# Autodesk Inventor assembly: złożenie
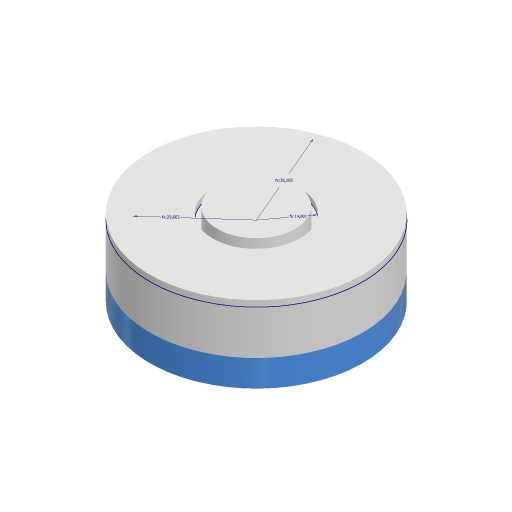
[picture p0: Inventor's stored thumbnail of the model, 512x512]
Saved by Autodesk Inventor 2024 (Build 280153000, 153)
## iProperties
Created: 2024-12-22
Part Number: złożenie
Document SubType Name: Assembly
Designer: Wicek
Author: Wicek
## Documents named in this file (8)
- I:\Dyski współdzielone\skill.ed TaskHunter\Model 3D\Przekładnia cykloidalna\złożenie.iam
- I:\Dyski współdzielone\skill.ed TaskHunter\Model 3D\Przekładnia cykloidalna\Korpus.ipt
- C:\Users\Wicek\OneDrive\Dokumenty\Inventor\Content Center Files\R2024\pl-PL\BS 290 SKF(09)\BS 290 SKF - SKF 608-2Z.ipt
- I:\Dyski współdzielone\skill.ed TaskHunter\Model 3D\Przekładnia cykloidalna\Dysk_we.ipt
- I:\Dyski współdzielone\skill.ed TaskHunter\Model 3D\Przekładnia cykloidalna\rotor.ipt
- I:\Dyski współdzielone\skill.ed TaskHunter\Model 3D\Przekładnia cykloidalna\Dysk_wy.ipt
- I:\Dyski współdzielone\skill.ed TaskHunter\Model 3D\Przekładnia cykloidalna\Korpus 2.ipt
- I:\Dyski współdzielone\skill.ed TaskHunter\Model 3D\Przekładnia cykloidalna\parametry.xlsx
## Components (7 placed, 6 different names)
1. Korpus:1 — Zestawiające:1, Zestawiające:4, Zestawiające:14
2. BS 290 SKF- osłonięte obustronnie SKF 608-2Z:1 — Zestawiające:2, Zestawiające:3, Równoległe:2, Zestawiające:4, Zestawiające:11, Zestawiające:12
3. Dysk_we:1 — Zestawiające:2, Zestawiające:1, Obrót:1, Zestawiające:6, Zestawiające:7, Zestawiające:12
4. rotor:1 — Zestawiające:3, Równoległe:2, Obrót:1, Obrót:2
5. Dysk_wy:1 — Zestawiające:8, Zestawiające:9, Zestawiające:10, Obrót:2, Zestawiające:13
6. BS 290 SKF- osłonięte obustronnie SKF 608-2Z:2 — Zestawiające:6, Zestawiające:7, Zestawiające:8, Zestawiające:9, Zestawiające:10, Zestawiające:11
7. Korpus 2:1 — Zestawiające:13, Zestawiające:14
## Relationships (16: Mate 13, RelateRotation 2, Flush 1)
- Zestawiające:1 [Mate]: Korpus:1 ↔ Dysk_we:1
- Zestawiające:2 [Mate]: BS 290 SKF- osłonięte obustronnie SKF 608-2Z:1 ↔ Dysk_we:1
- Zestawiające:3 [Mate]: BS 290 SKF- osłonięte obustronnie SKF 608-2Z:1 ↔ rotor:1
- Równoległe:2 [Flush]: BS 290 SKF- osłonięte obustronnie SKF 608-2Z:1 ↔ rotor:1
- Zestawiające:4 [Mate]: Korpus:1 ↔ BS 290 SKF- osłonięte obustronnie SKF 608-2Z:1
- Obrót:1 [RelateRotation] (0.0312 ul): Dysk_we:1 ↔ rotor:1
- Zestawiające:6 [Mate]: Dysk_we:1 ↔ BS 290 SKF- osłonięte obustronnie SKF 608-2Z:2
- Zestawiające:7 [Mate]: Dysk_we:1 ↔ BS 290 SKF- osłonięte obustronnie SKF 608-2Z:2
- Zestawiające:8 [Mate]: Dysk_wy:1 ↔ BS 290 SKF- osłonięte obustronnie SKF 608-2Z:2
- Zestawiające:9 [Mate]: Dysk_wy:1 ↔ BS 290 SKF- osłonięte obustronnie SKF 608-2Z:2
- Zestawiające:10 [Mate]: Dysk_wy:1 ↔ BS 290 SKF- osłonięte obustronnie SKF 608-2Z:2
- Zestawiające:11 [Mate]: BS 290 SKF- osłonięte obustronnie SKF 608-2Z:1 ↔ BS 290 SKF- osłonięte obustronnie SKF 608-2Z:2
- Obrót:2 [RelateRotation] (1 ul): rotor:1 ↔ Dysk_wy:1
- Zestawiające:12 [Mate]: BS 290 SKF- osłonięte obustronnie SKF 608-2Z:1 ↔ Dysk_we:1
- Zestawiające:13 [Mate]: Dysk_wy:1 ↔ Korpus 2:1
- Zestawiające:14 [Mate]: Korpus:1 ↔ Korpus 2:1
## Named parameters: Lrz = 11 mm, Lrw = 4 mm, Lh = 7 mm, N1 = 31, N2 = 6, Rr = 1.5 mm, R = 29.60282 mm, R1 = 5 mm, h1 = 2 mm, h2 = 5 mm, E1 = 0.75 mm, silnik_rw = 2.5 mm, silnik_r_wypust = 11 mm, silnik_d_srub = 31 mm, dwr1 = 4.2757 mm, dwr2 = 20.30141 mm, dwr = 29.60282 mm
